# Autodesk Inventor assembly: Assembly_Nema_Motor_attachement_for_XYstage
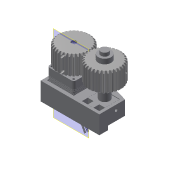
[picture p0: Inventor's stored thumbnail of the model, 180x180]
Saved by Autodesk Inventor 2019.4 (Build 234330000, 330)
## iProperties
Created: 2021-05-08
Part Number: Assembly_Nema_Motor_attachement_for_XYstage
Document SubType Name: Assembly
Designer: diederichbenedict
Author: diederichbenedict
## Documents named in this file (7)
- C:\Users\diederichbenedict\Dropbox\Dokumente\Promotion\PROJECTS\UC2\02_CAD\INVENTOR\uc2_v3\Assembly_Nema_Motor_attachement_for_XYstage.iam
- C:\Users\diederichbenedict\Dropbox\Dokumente\Promotion\PROJECTS\UC2\02_CAD\INVENTOR\uc2_v3\00_NEMA11.ipt
- C:\Users\diederichbenedict\Dropbox\Dokumente\Promotion\PROJECTS\UC2\02_CAD\INVENTOR\uc2_v3\00_micrometer_xy-stage.ipt
- C:\Users\diederichbenedict\Dropbox\Dokumente\Promotion\PROJECTS\UC2\02_CAD\INVENTOR\uc2_v3\cellstrom\cellSTORM_UC2_motorized_micrometer_gear2.ipt
- C:\Users\diederichbenedict\Dropbox\Dokumente\Promotion\PROJECTS\UC2\02_CAD\INVENTOR\uc2_v3\cellstrom\cellSTORM_UC2_motorized_micrometer_gear1.ipt
- C:\Users\diederichbenedict\Dropbox\Dokumente\Promotion\PROJECTS\UC2\02_CAD\INVENTOR\uc2_v3\00_micrometer_moun_xystage_china.ipt
- C:\Users\diederichbenedict\Dropbox\Dokumente\Promotion\PROJECTS\UC2\02_CAD\INVENTOR\uc2_v3\30_Mount_Nema_Motor_attachement_for_XYstage_v3.ipt
## Components (6 placed, 5 different names)
1. 00_NEMA11:1 — Mate:3, Insert:1, Angle:1, Angle:2, Flush:2, Angle:3, Flush:3, Flush:4
2. Spur Gear2:2 — Insert:1, Tangent:1
3. 00_micrometer_xy-stage:1 — Insert:2, Angle:2, Flush:2, Insert:3
4. Spur Gear2:3 — Tangent:1, Insert:2
5. 00_micrometer_moun_xystage_china:1 — Insert:3, Angle:3, Flush:3
6. 30_Mount_Nema_Motor_attachement_for_XYstage_v3:1 — Flush:4
## Relationships (11: Insert 3, Angle 3, Flush 3, Mate 1, Tangent 1)
- Mate:3: 00_NEMA11:1
- Insert:1: 00_NEMA11:1 ↔ Spur Gear2:2
- Tangent:1 (3 mm): Spur Gear2:2 ↔ Spur Gear2:3
- Angle:1 (180 deg): 00_NEMA11:1
- Insert:2 (-5 mm): 00_micrometer_xy-stage:1 ↔ Spur Gear2:3
- Angle:2 (0 deg): 00_NEMA11:1 ↔ 00_micrometer_xy-stage:1
- Flush:2: 00_NEMA11:1 ↔ 00_micrometer_xy-stage:1
- Insert:3: 00_micrometer_xy-stage:1 ↔ 00_micrometer_moun_xystage_china:1
- Angle:3 (0 deg): 00_NEMA11:1 ↔ 00_micrometer_moun_xystage_china:1
- Flush:3 (3 mm): 00_NEMA11:1 ↔ 00_micrometer_moun_xystage_china:1
- Flush:4: 00_NEMA11:1 ↔ 30_Mount_Nema_Motor_attachement_for_XYstage_v3:1
